# Autodesk Inventor assembly: StationDividerNoArm-ver1-1111-2021
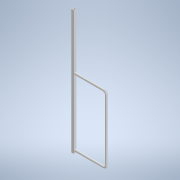
[picture p0: Inventor's stored thumbnail of the model, 180x180]
Saved by Autodesk Inventor 2021 (Build 250183000, 183)
## iProperties
Created: 2021-03-02
Part Number: StationDividerNoArm-ver1-1111-2021
Document SubType Name: Assembly
Designer: CMurray
Author: CMurray
## Documents named in this file (3)
- F:\PHRC CADD 2021\2021 Game Design Challenge\Player Station\Parts\StationDividerNoArm-ver1-1111-2021.iam
- F:\PHRC CADD 2021\2021 Game Design Challenge\Player Station\Parts\StationDividerPost-ver1-1111-2021.ipt
- F:\PHRC CADD 2021\2021 Game Design Challenge\Player Station\Parts\StationDividerBend-ver1-1111-2021.ipt
## Components (2 placed, 2 different names)
1. StationDividerPost-ver1-1111-2021:1 — Mate:1, Flush:1
2. StationDividerBend-ver1-1111-2021:1 — Mate:1, Flush:1
## Relationships (2: Mate 1, Flush 1)
- Mate:1: StationDividerPost-ver1-1111-2021:1 ↔ StationDividerBend-ver1-1111-2021:1
- Flush:1 (25.4 mm): StationDividerPost-ver1-1111-2021:1 ↔ StationDividerBend-ver1-1111-2021:1
